# Autodesk Inventor assembly: FullAssembly
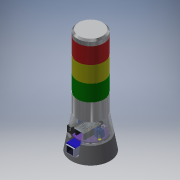
[picture p0: Inventor's stored thumbnail of the model, 180x180]
Saved by Autodesk Inventor 2018 (Build 220112000, 112)
## iProperties
Created: 2017-04-10
Part Number: FullAssembly
Document SubType Name: Assembly
Designer: dkt01
Author: dkt01
## Documents named in this file (5)
- C:\Users\dktur\Dropbox\StackLightMonitor\CAD\FullAssembly.iam
- C:\Users\dktur\Dropbox\StackLightMonitor\CAD\stackLight.iam
- C:\Users\dktur\Dropbox\StackLightMonitor\CAD\baseTop.ipt
- C:\Users\dktur\Dropbox\StackLightMonitor\CAD\ElectricalAssembly.iam
- C:\Users\dktur\Dropbox\StackLightMonitor\CAD\baseBottom.ipt
## Components (4 placed, 4 different names)
1. stackLight:1 [sub-assembly] — Insert:1, Insert:2
2. baseTop:1 — Insert:1, Insert:2, Mate:1, Mate:2, Insert:3
3. ElectricalAssembly:1 [sub-assembly] — Mate:1, Mate:2
4. baseBottom:1 — Insert:3
## Relationships (5: Insert 3, Mate 2)
- Insert:1: stackLight:1 ↔ baseTop:1
- Insert:2: stackLight:1 ↔ baseTop:1
- Mate:1: baseTop:1 ↔ ElectricalAssembly:1
- Mate:2: baseTop:1 ↔ ElectricalAssembly:1
- Insert:3: baseTop:1 ↔ baseBottom:1
